# Autodesk Inventor assembly: base plate w supports(1)
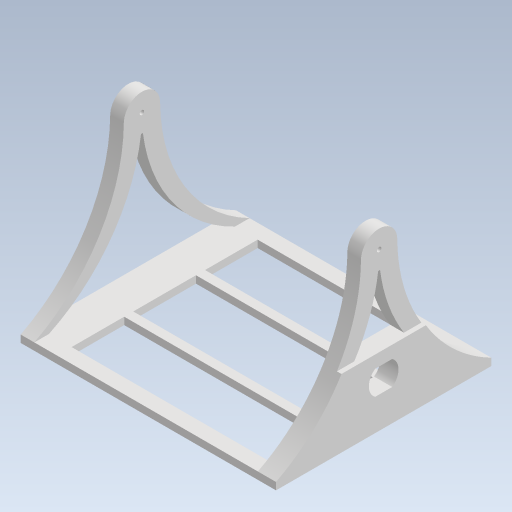
[picture p0: Inventor's stored thumbnail of the model, 512x512]
Saved by Autodesk Inventor 2023 (Build 270158000, 158)
## iProperties
Created: 2023-03-30
Part Number: base plate w supports(1)
Document SubType Name: Assembly
Designer: dverd
Author: dverd
## Documents named in this file (3)
- C:\Users\dverd\OneDrive\Documents\ME\ME 354\turbine lab 2.0\CAD\base plate w supports(1).iam
- C:\Users\dverd\OneDrive\Documents\ME\ME 354\turbine lab 2.0\CAD\base plate main.ipt
- C:\Users\dverd\OneDrive\Documents\ME\ME 354\turbine lab 2.0\CAD\rod support main.ipt
## Components (2 placed, 2 different names)
1. base plate main:1 — Mate:1, Mate:2, Flush:1
2. rod support main:1 — Mate:1, Mate:2, Flush:1
## Relationships (3: Mate 2, Flush 1)
- Mate:1: base plate main:1 ↔ rod support main:1
- Mate:2: base plate main:1 ↔ rod support main:1
- Flush:1: base plate main:1 ↔ rod support main:1
